# Autodesk Inventor assembly: rightBackWing
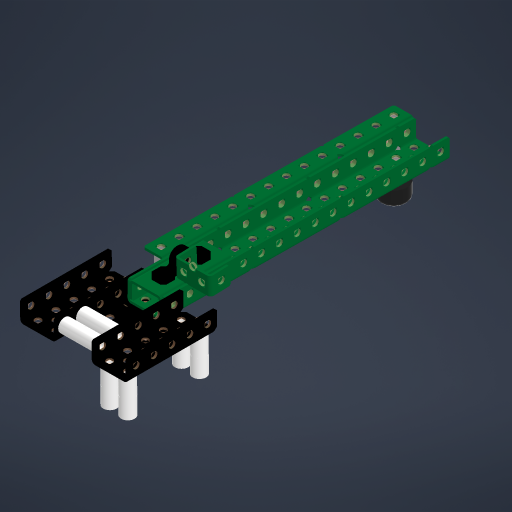
[picture p0: Inventor's stored thumbnail of the model, 512x512]
Saved by Autodesk Inventor 2023.4 (Build 274418000, 418)
## iProperties
Created: 2023-12-19
Part Number: rightBackWing
Document SubType Name: Assembly
Designer: Meer
Author: Meer
## Documents named in this file (12)
- C:\Users\Meer\OneDrive\Documents\GitHub\2024-599Z\Cad\NEW Wings\rightBackWing.iam
- C:\Users\Meer\OneDrive\Documents\GitHub\2024-599Z\Cad\Library\VEX-CAD-Inventor-1.4.0\Structure\Gussets\C Channel Coupler.ipt
- C:\Users\Meer\OneDrive\Documents\GitHub\2024-599Z\Cad\Library\VEX-CAD-Inventor-1.4.0\Structure\C Channel\Aluminum 1x2x1\Alu C 1x2x1x16.ipt
- C:\Users\Meer\OneDrive\Documents\GitHub\2024-599Z\Cad\Library\VEX-CAD-Inventor-1.4.0\Motion\Shaft LS\LS Pillow Bearing Block.ipt
- C:\Users\Meer\OneDrive\Documents\GitHub\2024-599Z\Cad\Library\VEX-CAD-Inventor-1.4.0\Structure\C Channel\Aluminum 1x2x1\Alu C 1x2x1x5.ipt
- C:\Users\Meer\OneDrive\Documents\GitHub\2024-599Z\Cad\Library\VEX-CAD-Inventor-1.4.0\Motion\Spacers\Spacer Nylon .313 OD\NSpacer .313 OD x .500.ipt
- C:\Users\Meer\OneDrive\Documents\GitHub\2024-599Z\Cad\Library\VEX-CAD-Inventor-1.4.0\Motion\Spacers\Spacer Nylon .313 OD.ipt
- C:\Users\Meer\OneDrive\Documents\GitHub\2024-599Z\Cad\Library\VEX-CAD-Inventor-1.4.0\Structure\C Channel\Aluminum 1x2x1\Alu C 1x2x1x1.ipt
- C:\Users\Meer\OneDrive\Documents\GitHub\2024-599Z\Cad\Library\VEX-CAD-Inventor-1.4.0\Structure\C Channel\Aluminum 1x3x1 Half\Alu C Half 1x3x1x14.ipt
- C:\Users\Meer\OneDrive\Documents\GitHub\2024-599Z\Cad\Library\VEX-CAD-Inventor-1.4.0\Structure\Standoff\Standoff 1.50.ipt
- C:\Users\Meer\OneDrive\Documents\GitHub\2024-599Z\Cad\Library\VEX-CAD-Inventor-1.4.0\Structure\Standoff.ipt
- C:\Users\Meer\OneDrive\Documents\GitHub\2024-599Z\Cad\Library\VEX-CAD-Inventor-1.4.0\Structure\Hardware\Rubber Bumper Threaded.ipt
## Components (24 placed, 9 different names)
1. C Channel Coupler:1
2. Alu C 1x2x1x16:1
3. LS Pillow Bearing Block:1
4. Alu C 1x2x1x5:1
5. NSpacer .313 OD x .500:1
6. NSpacer .313 OD x .500:2
7. NSpacer .313 OD x .500:3
8. NSpacer .313 OD x .500:4
9. Alu C 1x2x1x5:2
10. NSpacer .313 OD x .500:5
11. NSpacer .313 OD x .500:6
12. NSpacer .313 OD x .500:7
13. NSpacer .313 OD x .500:8
14. NSpacer .313 OD x .500:9
15. NSpacer .313 OD x .500:10
16. NSpacer .313 OD x .500:11
17. NSpacer .313 OD x .500:12
18. Alu C 1x2x1x1:1
19. C Channel Coupler:2
20. Alu C Half 1x3x1x14:1 — Insert:24, Insert:25
21. Standoff 1.50:1 — Insert:24
22. Rubber Bumper Threaded:1
23. Standoff 1.50:2 — Insert:25
24. Rubber Bumper Threaded:2
## Relationships (27: Insert 25, Mate 2)
- [Insert]: C Channel Coupler:1 ↔ Alu C 1x2x1x16:1
- [Mate]: C Channel Coupler:1 ↔ LS Pillow Bearing Block:1
- [Insert]: NSpacer .313 OD x .500:1 ↔ NSpacer .313 OD x .500:2
- [Insert]: NSpacer .313 OD x .500:3 ↔ NSpacer .313 OD x .500:4
- [Insert]: NSpacer .313 OD x .500:1 ↔ Alu C 1x2x1x5:2
- [Insert]: NSpacer .313 OD x .500:3 ↔ Alu C 1x2x1x5:2
- [Insert]: NSpacer .313 OD x .500:5 ↔ NSpacer .313 OD x .500:6
- [Insert]: Alu C 1x2x1x5:2 ↔ NSpacer .313 OD x .500:5
- [Insert]: NSpacer .313 OD x .500:7 ↔ NSpacer .313 OD x .500:8
- [Insert]: Alu C 1x2x1x5:2 ↔ NSpacer .313 OD x .500:8
- [Insert]: Alu C 1x2x1x5:2 ↔ NSpacer .313 OD x .500:5
- [Insert]: NSpacer .313 OD x .500:11 ↔ NSpacer .313 OD x .500:12
- [Insert]: NSpacer .313 OD x .500:9 ↔ NSpacer .313 OD x .500:10
- [Insert]: Alu C 1x2x1x5:2 ↔ NSpacer .313 OD x .500:11
- [Insert]: Alu C 1x2x1x5:1 ↔ NSpacer .313 OD x .500:12
- [Insert]: Alu C 1x2x1x5:1 ↔ NSpacer .313 OD x .500:10
- [Insert]: Alu C 1x2x1x5:2 ↔ NSpacer .313 OD x .500:9
- [Insert]: Alu C 1x2x1x16:1 ↔ Alu C 1x2x1x5:1
- [Mate]: C Channel Coupler:1 ↔ Alu C 1x2x1x16:1
- [Insert]: C Channel Coupler:1 ↔ LS Pillow Bearing Block:1
- [Insert]: LS Pillow Bearing Block:1 ↔ Alu C 1x2x1x1:1
- [Insert]: Alu C 1x2x1x16:1 ↔ Alu C Half 1x3x1x14:1
- [Insert]: Alu C 1x2x1x16:1 ↔ Alu C Half 1x3x1x14:1
- [Insert]: Standoff 1.50:1 ↔ Rubber Bumper Threaded:1
- [Insert]: Standoff 1.50:2 ↔ Rubber Bumper Threaded:2
- Insert:24: Alu C Half 1x3x1x14:1 ↔ Standoff 1.50:1
- Insert:25: Alu C Half 1x3x1x14:1 ↔ Standoff 1.50:2
## Named parameters: d1362_d1343 = 0 mm, d1363_d1345 = 0 mm, d1364_d1347 = 0 mm, d1365_d1348 = 0 mm, d1366_d1349_d1345 = 0 mm, d1367_d1350 = 0 mm, d1368_d1351_d1345 = 0 mm, d1369_d1353 = 0 mm, d1370_d1354 = 0 mm, d1371_d1355 = 0 mm, d1374_d1358 = 0 mm, d26_d27 = 0 mm
